# Autodesk Inventor assembly: Chest
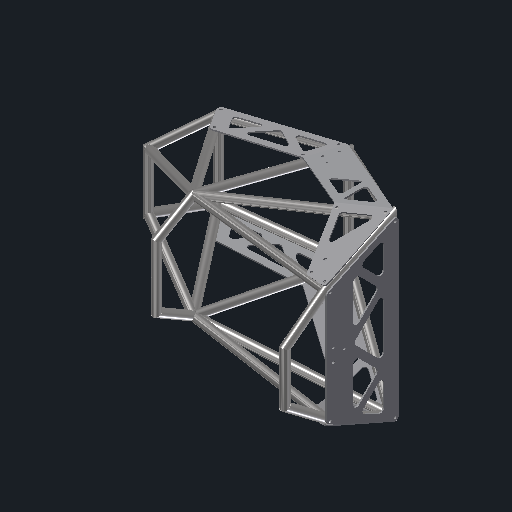
[picture p0: Inventor's stored thumbnail of the model, 512x512]
Saved by Autodesk Inventor 2025.2 (Build 292293000, 293)
## iProperties
Created: 2025-02-15
Part Number: Chest
Document SubType Name: Assembly
Designer: valer
_SolveAssemblyDoc: Frame Generator Solve Assembly
_Version: 25.0.0
Author: valer
## Documents named in this file (6)
- C:\Users\valer\Desktop\str1ker\cad\Chest.iam
- C:\Users\valer\Desktop\str1ker\cad\ChestFrame.ipt
- C:\Users\valer\Desktop\str1ker\cad\ChestFrame.iam
- C:\Users\valer\Desktop\str1ker\cad\ChestFront.ipt
- C:\Users\valer\Desktop\str1ker\cad\ChestSide.ipt
- C:\Users\valer\Desktop\str1ker\cad\ChestSideMirror.ipt
## Components (5 placed, 4 different names)
1. ChestFrame:1 — Flush:1, Flush:2, Mate:1, Flush:3, Mate:2, Mate:3, Mate:4, Mate:7, Mate:8, Mate:9, Mate:10, Mate:11, Mate:12, Mate:13, Mate:14
2. ChestFrame:2 [sub-assembly]
3. ChestFront:1 — Mate:2, Mate:3, Mate:4
4. ChestSide:1 — Mate:7, Mate:8, Mate:9, Mate:10, Mate:11
5. ChestSideMirror:1 — Mate:12, Mate:13, Mate:14
## Relationships (15: Mate 12, Flush 3)
- Flush:1: ChestFrame:1
- Flush:2: ChestFrame:1
- Mate:1: ChestFrame:1
- Flush:3: ChestFrame:1
- Mate:2: ChestFrame:1 ↔ ChestFront:1
- Mate:3: ChestFrame:1 ↔ ChestFront:1
- Mate:4 (9.525 mm): ChestFrame:1 ↔ ChestFront:1
- Mate:7 (11.1125 mm): ChestFrame:1 ↔ ChestSide:1
- Mate:8: ChestFrame:1 ↔ ChestSide:1
- Mate:9: ChestFrame:1 ↔ ChestSide:1
- Mate:10: ChestFrame:1 ↔ ChestSide:1
- Mate:11: ChestFrame:1 ↔ ChestSide:1
- Mate:12 (11.1125 mm): ChestFrame:1 ↔ ChestSideMirror:1
- Mate:13: ChestFrame:1 ↔ ChestSideMirror:1
- Mate:14: ChestFrame:1 ↔ ChestSideMirror:1
